# Autodesk Inventor assembly: SLIM_ASSEMBLED
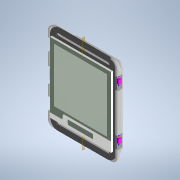
[picture p0: Inventor's stored thumbnail of the model, 180x180]
Saved by Autodesk Inventor 2020 (Build 240168000, 168)
## iProperties
Created: 2021-08-24
Part Number: SLIM_ASSEMBLED
Document SubType Name: Assembly
Designer: nigel
Author: nigel
## Documents named in this file (3)
- D:\NIGEL\OneDrive - Singapore University of Technology and Design\3D Objects\Watchy\CAD\Cases\SlimV2\SLIM_ASSEMBLED.iam
- D:\NIGEL\OneDrive - Singapore University of Technology and Design\3D Objects\Watchy\CAD\Cases\SlimV2\Bottom.ipt
- D:\NIGEL\OneDrive - Singapore University of Technology and Design\3D Objects\Watchy\CAD\Base Model\WATCHY.iam
## Components (2 placed, 2 different names)
1. Bottom:1 — Flush:1, Flush:2, Flush:3
2. WATCHY:1 [sub-assembly] — Flush:1, Flush:2, Flush:3
## Relationships (3: Flush 3)
- Flush:1: Bottom:1 ↔ WATCHY:1
- Flush:2: Bottom:1 ↔ WATCHY:1
- Flush:3: Bottom:1 ↔ WATCHY:1
